# Autodesk Inventor assembly: Gripper_Link_Holder
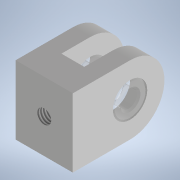
[picture p0: Inventor's stored thumbnail of the model, 180x180]
Saved by Autodesk Inventor 2021.3 (Build 253353000, 353)
## iProperties
Created: 2021-04-16
Part Number: Gripper_Link_Holder
Document SubType Name: Assembly
Designer: domin
Author: domin
## Documents named in this file (3)
- E:\Transfer\Sync\Hivemind\1-MCI-Unterlagen\Master\Semester 2\Projekt 1\Hausberger\Workfolder_Dommy\Gripper\Gripper_Link_Holder.iam
- E:\Transfer\Sync\Hivemind\1-MCI-Unterlagen\Master\Semester 2\Projekt 1\Hausberger\Workfolder_Dommy\Gripper\Gripper_Link_Holder.ipt
- E:\Transfer\Sync\Hivemind\1-MCI-Unterlagen\Master\Semester 2\Projekt 1\Hausberger\Workfolder_Dommy\Gripper\Zukauf\Gleitlager\TFZB3-3.ipt
## Components (3 placed, 2 different names)
1. Gripper_Link_Holder:1 — Mate:1, Mate:2, Mate:3, Mate:4, Mate:5, Mate:6, Flush:1
2. TFZB3-3:1 — Mate:4, Flush:1, Angle:1
3. TFZB3-3:2 — Mate:5, Mate:6, Angle:2
## Relationships (9: Mate 6, Angle 2, Flush 1)
- Mate:1: Gripper_Link_Holder:1
- Mate:2: Gripper_Link_Holder:1
- Mate:3: Gripper_Link_Holder:1
- Mate:4: Gripper_Link_Holder:1 ↔ TFZB3-3:1
- Mate:5: Gripper_Link_Holder:1 ↔ TFZB3-3:2
- Mate:6: Gripper_Link_Holder:1 ↔ TFZB3-3:2
- Flush:1: Gripper_Link_Holder:1 ↔ TFZB3-3:1
- Angle:1 (0 deg): TFZB3-3:1
- Angle:2 (0 deg): TFZB3-3:2
